# Autodesk Inventor assembly: Assembly
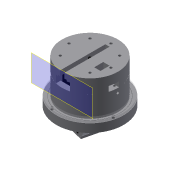
[picture p0: Inventor's stored thumbnail of the model, 180x180]
Saved by Autodesk Inventor 2018 (Build 220112000, 112)
## iProperties
Created: 2017-12-03
Part Number: Assembly
Document SubType Name: Assembly
Designer: Bardo91
Author: Bardo91
## Documents named in this file (8)
- C:\Users\Bardo91\Desktop\hecatonquiros\cad_models\arm_3_dog\serial_model\Assembly.iam
- C:\Users\Bardo91\Desktop\hecatonquiros\cad_models\arm_3_dog\serial_model\arm_0_attachment.ipt
- C:\Users\Bardo91\Desktop\hecatonquiros\cad_models\arm_3_dog\serial_model\arm_0_top.ipt
- C:\Users\Bardo91\Desktop\hecatonquiros\cad_models\arm_3_dog\serial_model\servo_FT_SC.ipt
- C:\Users\Bardo91\Desktop\hecatonquiros\cad_models\arm_3_dog\serial_model\arm_0_bottom.ipt
- C:\Users\Bardo91\Desktop\hecatonquiros\cad_models\arm_3_dog\serial_model\arm_0_bottom_top_lock.ipt
- C:\Users\Bardo91\Desktop\hecatonquiros\cad_models\arm_3_dog\serial_model\servo_FT_SC_horn_1.ipt
- C:\Users\Bardo91\Desktop\hecatonquiros\cad_models\arm_3_dog\serial_model\arm_0_bottom_case.ipt
## Components (8 placed, 7 different names)
1. arm_0_attachment:1 — Mate:1, Mate:2, Mate:3
2. arm_0_top:1 — Mate:1, Mate:2, Mate:3, Mate:4, Mate:5, Mate:6, Mate:7, Flush:1
3. servo_FT_SC:1 — Mate:4, Mate:5, Mate:6, Mate:17, Mate:18
4. servo_FT_SC_horn_1:1 — Mate:17, Mate:18, Mate:19, Mate:20
5. arm_0_bottom:1 — Mate:7, Flush:1, Mate:14, Mate:15, Mate:16, Mate:19, Mate:20, Mate:21, Mate:22, Mate:23, Mate:24, Mate:25, Mate:26, Mate:27
6. arm_0_bottom_top_lock:1 — Mate:14, Mate:15, Mate:16
7. servo_FT_SC:2 — Mate:21, Mate:22, Mate:23
8. arm_0_bottom_case:1 — Mate:24, Mate:25, Mate:26, Mate:27
## Relationships (22: Mate 21, Flush 1)
- Mate:1: arm_0_attachment:1 ↔ arm_0_top:1
- Mate:2: arm_0_attachment:1 ↔ arm_0_top:1
- Mate:3: arm_0_attachment:1 ↔ arm_0_top:1
- Mate:4: arm_0_top:1 ↔ servo_FT_SC:1
- Mate:5: arm_0_top:1 ↔ servo_FT_SC:1
- Mate:6: arm_0_top:1 ↔ servo_FT_SC:1
- Mate:7: arm_0_top:1 ↔ arm_0_bottom:1
- Flush:1: arm_0_top:1 ↔ arm_0_bottom:1
- Mate:14: arm_0_bottom:1 ↔ arm_0_bottom_top_lock:1
- Mate:15: arm_0_bottom:1 ↔ arm_0_bottom_top_lock:1
- Mate:16: arm_0_bottom:1 ↔ arm_0_bottom_top_lock:1
- Mate:17: servo_FT_SC:1 ↔ servo_FT_SC_horn_1:1
- Mate:18: servo_FT_SC:1 ↔ servo_FT_SC_horn_1:1
- Mate:19: servo_FT_SC_horn_1:1 ↔ arm_0_bottom:1
- Mate:20: servo_FT_SC_horn_1:1 ↔ arm_0_bottom:1
- Mate:21: arm_0_bottom:1 ↔ servo_FT_SC:2
- Mate:22: arm_0_bottom:1 ↔ servo_FT_SC:2
- Mate:23: arm_0_bottom:1 ↔ servo_FT_SC:2
- Mate:24: arm_0_bottom:1 ↔ arm_0_bottom_case:1
- Mate:25: arm_0_bottom:1 ↔ arm_0_bottom_case:1
- Mate:26: arm_0_bottom:1 ↔ arm_0_bottom_case:1
- Mate:27: arm_0_bottom:1 ↔ arm_0_bottom_case:1
